# Autodesk Inventor assembly: montaje carro x lado polea
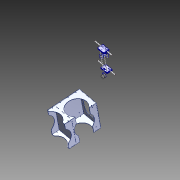
[picture p0: Inventor's stored thumbnail of the model, 180x180]
Saved by Autodesk Inventor 2012 SP2 (Build 160219200, 219)
## iProperties
Created: 2014-06-29
Part Number: montaje carro x lado polea
Document SubType Name: Assembly
Designer: Principal
Author: Principal
## Documents named in this file (24)
- E:\descargas\Archivos replicatorg\rockstar mini\impresora juan marc albert\montaje carro x lado polea.iam
- E:\descargas\Archivos replicatorg\rockstar mini\impresora juan marc albert\cojinete lm10uu.ipt
- E:\descargas\Archivos replicatorg\rockstar mini\impresora juan marc albert\varilla 10 carro x.ipt
- E:\descargas\Archivos replicatorg\rockstar mini\impresora juan marc albert\carro x lado motor pieza 1.ipt
- E:\descargas\Archivos replicatorg\rockstar mini\impresora juan marc albert\carro x lado motor pieza 2.ipt
- E:\descargas\Archivos replicatorg\rockstar mini\impresora juan marc albert\carro x lado motor pieza 3.ipt
- E:\descargas\Archivos replicatorg\rockstar mini\impresora juan marc albert\carro x lado motor pieza 4.ipt
- E:\descargas\Archivos replicatorg\rockstar mini\impresora juan marc albert\Motor_NEMA17.ipt
- E:\descargas\Archivos replicatorg\rockstar mini\impresora juan marc albert\carro x lado motor pieza 5 soporte nema.ipt
- E:\descargas\Archivos replicatorg\rockstar mini\impresora juan marc albert\polea gt2 20 diente.ipt
- E:\descargas\Archivos replicatorg\rockstar mini\impresora juan marc albert\varilla 10 carro y.ipt
- E:\descargas\Archivos replicatorg\rockstar mini\impresora juan marc albert\brida correas eje y.ipt
- E:\descargas\Archivos replicatorg\rockstar mini\impresora juan marc albert\carro x lado polea pieza1.ipt
- E:\descargas\Archivos replicatorg\rockstar mini\impresora juan marc albert\carro x lado polea pieza2.ipt
- E:\descargas\Archivos replicatorg\rockstar mini\impresora juan marc albert\carro x lado polea pieza3.ipt
- E:\descargas\Archivos replicatorg\rockstar mini\impresora juan marc albert\carro x lado polea pieza4 tapa.ipt
- E:\descargas\Archivos replicatorg\rockstar mini\impresora juan marc albert\tapa polea x.ipt
- E:\descargas\Archivos replicatorg\rockstar mini\impresora juan marc albert\tapa polea x 2.ipt
- E:\descargas\Archivos replicatorg\rockstar mini\impresora juan marc albert\soporte polea eje x.ipt
- E:\descargas\Archivos replicatorg\rockstar mini\impresora juan marc albert\eje polea x.ipt
- E:\descargas\Archivos replicatorg\rockstar mini\impresora juan marc albert\cojinete polea x.ipt
- E:\descargas\Archivos replicatorg\rockstar mini\impresora juan marc albert\archivos step\Componentes importados\CONJUNT ESFERA INT\CONJUNT ESFERA INT.iam
- E:\descargas\Archivos replicatorg\rockstar mini\impresora juan marc albert\plataforma extrusor.ipt
- E:\descargas\Archivos replicatorg\rockstar mini\impresora juan marc albert\mk7 extrusor.iam
## Components (46 placed, 23 different names)
1. brida correas eje y:1 — Nivelación:5, Coincidencia:17, Coincidencia:18
2. brida correas eje y:2 — Nivelación:4, Coincidencia:19, Coincidencia:20
3. brida correas eje y:3 — Nivelación:3, Coincidencia:12, Coincidencia:13
4. brida correas eje y:4 — Nivelación:2, Coincidencia:11, Coincidencia:14
5. carro x lado motor pieza 1:1 — Insertar:1, Insertar:2, Insertar:7, Insertar:8, Nivelación:2, Nivelación:3, Coincidencia:11, Coincidencia:12, Coincidencia:13, Coincidencia:14, Tangente:4
6. carro x lado motor pieza 2:1 — Insertar:1, Insertar:2, Insertar:3, Insertar:4, Insertar:17, Insertar:18, Coincidencia:31
7. carro x lado motor pieza 2:2 — Insertar:3, Insertar:4, Insertar:5, Insertar:6, Coincidencia:32
8. carro x lado motor pieza 2:3 — Insertar:5, Insertar:6, Insertar:13, Insertar:14
9. carro x lado motor pieza 3:1 — Insertar:7, Insertar:8, Insertar:9, Insertar:10
10. carro x lado motor pieza 3:2 — Insertar:9, Insertar:10, Insertar:11, Insertar:12
11. carro x lado motor pieza 3:3 — Insertar:11, Insertar:12
12. carro x lado motor pieza 4:1 — Insertar:13, Insertar:14, Nivelación:1, Coincidencia:9, Coincidencia:10, Tangente:1, Tangente:2, Tangente:3
13. carro x lado motor pieza 5 soporte nema:1 — Insertar:15, Insertar:16, Nivelación:1, Coincidencia:9, Coincidencia:10
14. Motor_NEMA17:1 — Insertar:15, Insertar:16, Insertar:19
15. varilla 10 carro x:1 — Insertar:18, Insertar:51
16. varilla 10 carro x:2 — Insertar:17, Insertar:50
17. varilla 10 carro y:1 — Insertar:55
18. varilla 10 carro y:2 — Insertar:54
19. polea gt2 20 diente:1 — Insertar:19
20. carro x lado polea pieza1:1 — Insertar:26, Insertar:27, Nivelación:4, Nivelación:5, Coincidencia:17, Coincidencia:18, Coincidencia:19, Coincidencia:20, Insertar:39, Insertar:40, Insertar:52, Insertar:53
21. carro x lado polea pieza3:1 — Insertar:26, Insertar:27, Insertar:28, Insertar:29
22. carro x lado polea pieza3:2 — Insertar:28, Insertar:29, Insertar:30, Insertar:31
23. carro x lado polea pieza3:3 — Insertar:30, Insertar:31, Insertar:48
24. tapa polea x:1 — Coincidencia:25, Coincidencia:26, Nivelación:12, Nivelación:13, Nivelación:14, Coincidencia:27, Coincidencia:28, Nivelación:15, Nivelación:16, Insertar:52, Insertar:53
25. tapa polea x 2:1 — Coincidencia:24, Nivelación:11, Coincidencia:25, Nivelación:16
26. soporte polea eje x:1 — Insertar:35, Coincidencia:26, Nivelación:14, Coincidencia:28, Nivelación:15
27. eje polea x:1 — Insertar:37
28. cojinete polea x:1 — Insertar:36, Insertar:37
29. cojinete polea x:2 — Insertar:35, Insertar:38
30. polea gt2 20 diente:2 — Insertar:38
31. soporte polea eje x:2 — Insertar:36, Coincidencia:24, Nivelación:11, Nivelación:12, Nivelación:13, Coincidencia:27
32. carro x lado polea pieza2:4 — Insertar:39, Insertar:40, Insertar:41, Insertar:42, Insertar:43, Insertar:50, Insertar:51
33. carro x lado polea pieza2:5 — Insertar:41, Insertar:42, Insertar:43, Insertar:44, Insertar:45, Insertar:46, Coincidencia:29, Coincidencia:30
34. carro x lado polea pieza2:6 — Insertar:44, Insertar:45, Insertar:46, Insertar:47, Insertar:49
35. carro x lado polea pieza4 tapa:1 — Insertar:47, Insertar:48, Insertar:49, Tangente:5, Tangente:6, Tangente:7, Tangente:8, Insertar:58
36. cojinete lm10uu:1 — Coincidencia:32, Tangente:3, Tangente:4
37. cojinete lm10uu:2 — Coincidencia:29, Tangente:5, Tangente:6
38. cojinete lm10uu:3 — Coincidencia:30, Tangente:7, Tangente:8, Insertar:55
39. cojinete lm10uu:4 — Coincidencia:31, Tangente:1, Tangente:2, Insertar:54
40. CONJUNT ESFERA INT:1 [sub-assembly]
41. plataforma extrusor:1 — Coincidencia:33, Coincidencia:34, Coincidencia:35, Coincidencia:36, Tangente:9, Tangente:10, Tangente:11, Tangente:12, Tangente:13, Tangente:14, Tangente:15, Tangente:16, Nivelación:17, Coincidencia:37
42. cojinete lm10uu:5 — Coincidencia:33, Tangente:11, Tangente:13
43. cojinete lm10uu:6 — Coincidencia:34, Tangente:9, Tangente:16
44. cojinete lm10uu:7 — Coincidencia:35, Tangente:10, Tangente:15
45. cojinete lm10uu:8 — Coincidencia:36, Tangente:12, Tangente:14, Insertar:58
46. mk7 extrusor:1 [sub-assembly] — Nivelación:17, Coincidencia:37
## Relationships (99: Insert 47, Mate 24, Tangent 16, Flush 12)
- Insertar:1: carro x lado motor pieza 1:1 ↔ carro x lado motor pieza 2:1
- Insertar:2: carro x lado motor pieza 1:1 ↔ carro x lado motor pieza 2:1
- Insertar:3: carro x lado motor pieza 2:1 ↔ carro x lado motor pieza 2:2
- Insertar:4: carro x lado motor pieza 2:1 ↔ carro x lado motor pieza 2:2
- Insertar:5: carro x lado motor pieza 2:2 ↔ carro x lado motor pieza 2:3
- Insertar:6: carro x lado motor pieza 2:2 ↔ carro x lado motor pieza 2:3
- Insertar:7: carro x lado motor pieza 1:1 ↔ carro x lado motor pieza 3:1
- Insertar:8: carro x lado motor pieza 1:1 ↔ carro x lado motor pieza 3:1
- Insertar:9: carro x lado motor pieza 3:1 ↔ carro x lado motor pieza 3:2
- Insertar:10: carro x lado motor pieza 3:1 ↔ carro x lado motor pieza 3:2
- Insertar:11: carro x lado motor pieza 3:2 ↔ carro x lado motor pieza 3:3
- Insertar:12: carro x lado motor pieza 3:2 ↔ carro x lado motor pieza 3:3
- Insertar:13: carro x lado motor pieza 2:3 ↔ carro x lado motor pieza 4:1
- Insertar:14: carro x lado motor pieza 2:3 ↔ carro x lado motor pieza 4:1
- Insertar:15: carro x lado motor pieza 5 soporte nema:1 ↔ Motor_NEMA17:1
- Insertar:16: carro x lado motor pieza 5 soporte nema:1 ↔ Motor_NEMA17:1
- Nivelación:1 [Flush]: carro x lado motor pieza 4:1 ↔ carro x lado motor pieza 5 soporte nema:1
- Coincidencia:9 [Mate]: carro x lado motor pieza 4:1 ↔ carro x lado motor pieza 5 soporte nema:1
- Coincidencia:10 [Mate]: carro x lado motor pieza 4:1 ↔ carro x lado motor pieza 5 soporte nema:1
- Nivelación:2 [Flush]: brida correas eje y:4 ↔ carro x lado motor pieza 1:1
- Nivelación:3 [Flush]: brida correas eje y:3 ↔ carro x lado motor pieza 1:1
- Coincidencia:11 [Mate]: brida correas eje y:4 ↔ carro x lado motor pieza 1:1
- Coincidencia:12 [Mate]: brida correas eje y:3 ↔ carro x lado motor pieza 1:1
- Coincidencia:13 [Mate]: brida correas eje y:3 ↔ carro x lado motor pieza 1:1
- Coincidencia:14 [Mate]: brida correas eje y:4 ↔ carro x lado motor pieza 1:1
- Insertar:17: carro x lado motor pieza 2:1 ↔ varilla 10 carro x:2
- Insertar:18: carro x lado motor pieza 2:1 ↔ varilla 10 carro x:1
- Insertar:19 (3 mm): Motor_NEMA17:1 ↔ polea gt2 20 diente:1
- Insertar:26: carro x lado polea pieza1:1 ↔ carro x lado polea pieza3:1
- Insertar:27: carro x lado polea pieza1:1 ↔ carro x lado polea pieza3:1
- Insertar:28: carro x lado polea pieza3:1 ↔ carro x lado polea pieza3:2
- Insertar:29: carro x lado polea pieza3:1 ↔ carro x lado polea pieza3:2
- Insertar:30: carro x lado polea pieza3:2 ↔ carro x lado polea pieza3:3
- Insertar:31: carro x lado polea pieza3:2 ↔ carro x lado polea pieza3:3
- Nivelación:4 [Flush]: brida correas eje y:2 ↔ carro x lado polea pieza1:1
- Nivelación:5 [Flush]: brida correas eje y:1 ↔ carro x lado polea pieza1:1
- Coincidencia:17 [Mate]: brida correas eje y:1 ↔ carro x lado polea pieza1:1
- Coincidencia:18 [Mate]: brida correas eje y:1 ↔ carro x lado polea pieza1:1
- Coincidencia:19 [Mate]: brida correas eje y:2 ↔ carro x lado polea pieza1:1
- Coincidencia:20 [Mate]: brida correas eje y:2 ↔ carro x lado polea pieza1:1
- Insertar:35: soporte polea eje x:1 ↔ cojinete polea x:2
- Insertar:36: cojinete polea x:1 ↔ soporte polea eje x:2
- Coincidencia:24 [Mate]: tapa polea x 2:1 ↔ soporte polea eje x:2
- Nivelación:11 [Flush]: tapa polea x 2:1 ↔ soporte polea eje x:2
- Insertar:37: eje polea x:1 ↔ cojinete polea x:1
- Insertar:38 (0.5 mm): cojinete polea x:2 ↔ polea gt2 20 diente:2
- Coincidencia:25 [Mate]: tapa polea x:1 ↔ tapa polea x 2:1
- Coincidencia:26 [Mate]: tapa polea x:1 ↔ soporte polea eje x:1
- Nivelación:12 [Flush]: tapa polea x:1 ↔ soporte polea eje x:2
- Nivelación:13 [Flush]: tapa polea x:1 ↔ soporte polea eje x:2
- Nivelación:14 [Flush]: tapa polea x:1 ↔ soporte polea eje x:1
- Coincidencia:27 [Mate]: tapa polea x:1 ↔ soporte polea eje x:2
- Coincidencia:28 [Mate]: tapa polea x:1 ↔ soporte polea eje x:1
- Nivelación:15 [Flush]: tapa polea x:1 ↔ soporte polea eje x:1
- Nivelación:16 [Flush]: tapa polea x:1 ↔ tapa polea x 2:1
- Insertar:39: carro x lado polea pieza1:1 ↔ carro x lado polea pieza2:4
- Insertar:40: carro x lado polea pieza1:1 ↔ carro x lado polea pieza2:4
- Insertar:41: carro x lado polea pieza2:4 ↔ carro x lado polea pieza2:5
- Insertar:42: carro x lado polea pieza2:4 ↔ carro x lado polea pieza2:5
- Insertar:43: carro x lado polea pieza2:4 ↔ carro x lado polea pieza2:5
- Insertar:44: carro x lado polea pieza2:5 ↔ carro x lado polea pieza2:6
- Insertar:45: carro x lado polea pieza2:5 ↔ carro x lado polea pieza2:6
- Insertar:46: carro x lado polea pieza2:5 ↔ carro x lado polea pieza2:6
- Insertar:47: carro x lado polea pieza2:6 ↔ carro x lado polea pieza4 tapa:1
- Insertar:48: carro x lado polea pieza3:3 ↔ carro x lado polea pieza4 tapa:1
- Insertar:49: carro x lado polea pieza2:6 ↔ carro x lado polea pieza4 tapa:1
- Insertar:50: varilla 10 carro x:2 ↔ carro x lado polea pieza2:4
- Insertar:51: varilla 10 carro x:1 ↔ carro x lado polea pieza2:4
- Insertar:52: carro x lado polea pieza1:1 ↔ tapa polea x:1
- Insertar:53: carro x lado polea pieza1:1 ↔ tapa polea x:1
- Coincidencia:29 [Mate]: carro x lado polea pieza2:5 ↔ cojinete lm10uu:2
- Coincidencia:30 [Mate]: carro x lado polea pieza2:5 ↔ cojinete lm10uu:3
- Coincidencia:31 [Mate]: carro x lado motor pieza 2:1 ↔ cojinete lm10uu:4
- Coincidencia:32 [Mate]: carro x lado motor pieza 2:2 ↔ cojinete lm10uu:1
- Tangente:1: carro x lado motor pieza 4:1 ↔ cojinete lm10uu:4
- Tangente:2: carro x lado motor pieza 4:1 ↔ cojinete lm10uu:4
- Tangente:3: carro x lado motor pieza 4:1 ↔ cojinete lm10uu:1
- Tangente:4: carro x lado motor pieza 1:1 ↔ cojinete lm10uu:1
- Tangente:5: carro x lado polea pieza4 tapa:1 ↔ cojinete lm10uu:2
- Tangente:6: carro x lado polea pieza4 tapa:1 ↔ cojinete lm10uu:2
- Tangente:7: carro x lado polea pieza4 tapa:1 ↔ cojinete lm10uu:3
- Tangente:8: carro x lado polea pieza4 tapa:1 ↔ cojinete lm10uu:3
- Insertar:54 (-125 mm): varilla 10 carro y:2 ↔ cojinete lm10uu:4
- Insertar:55 (-125 mm): varilla 10 carro y:1 ↔ cojinete lm10uu:3
- Coincidencia:33 [Mate]: plataforma extrusor:1 ↔ cojinete lm10uu:5
- Coincidencia:34 [Mate]: plataforma extrusor:1 ↔ cojinete lm10uu:6
- Coincidencia:35 [Mate]: plataforma extrusor:1 ↔ cojinete lm10uu:7
- Coincidencia:36 [Mate]: plataforma extrusor:1 ↔ cojinete lm10uu:8
- Tangente:9: plataforma extrusor:1 ↔ cojinete lm10uu:6
- Tangente:10: plataforma extrusor:1 ↔ cojinete lm10uu:7
- Tangente:11: plataforma extrusor:1 ↔ cojinete lm10uu:5
- Tangente:12: plataforma extrusor:1 ↔ cojinete lm10uu:8
- Tangente:13: plataforma extrusor:1 ↔ cojinete lm10uu:5
- Tangente:14: plataforma extrusor:1 ↔ cojinete lm10uu:8
- Tangente:15: plataforma extrusor:1 ↔ cojinete lm10uu:7
- Tangente:16: plataforma extrusor:1 ↔ cojinete lm10uu:6
- Insertar:58 (90 mm): carro x lado polea pieza4 tapa:1 ↔ cojinete lm10uu:8
- Nivelación:17 [Flush]: plataforma extrusor:1 ↔ mk7 extrusor:1
- Coincidencia:37 [Mate]: plataforma extrusor:1 ↔ mk7 extrusor:1
